# Autodesk Inventor assembly: ASY GBK предварительная торцевая
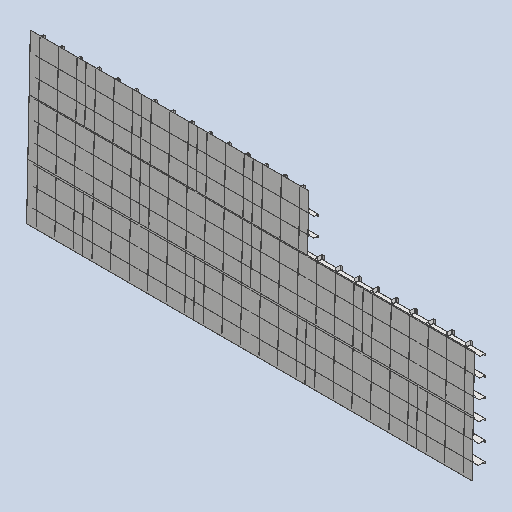
[picture p0: Inventor's stored thumbnail of the model, 512x512]
Saved by Autodesk Inventor 2026.2 (Build 302298000, 298)
## iProperties
Created: 2026-05-20
Part Number: ASY GBK предварительная торцевая
Document SubType Name: Assembly
Designer: admin
Mass: 2.96106e+06 g
Surface Area: 1.91261e+06 cm^2
Volume: 377205 cm^3
Density: 7.85 g/cm^3
Author: admin
## Documents named in this file (6)
- C:\Users\admin\Documents\Inventor\GBK-Gubkinskiy\ASY GBK предварительная торцевая.iam
- C:\Users\admin\Documents\Inventor\GBK-Gubkinskiy\ASY GBK 1110 long wall shield 1.iam
- C:\Users\admin\Documents\Inventor\GBK-Gubkinskiy\ASY GBK 1120 long wall shield 2.iam
- C:\Users\admin\Documents\Inventor\GBK-Gubkinskiy\ASY GBK 1210 long wall shield 3.iam
- C:\Users\admin\Documents\Inventor\GBK-Gubkinskiy\ASY GBK 1310 long wall shield 4.iam
- C:\Users\admin\Documents\Inventor\GBK-Gubkinskiy\08 ASY GBK wall shield 1.3.8.iam
## Components (14 placed, 5 different names)
1. ASY GBK 1110 long wall shield 1:1 [sub-assembly]
2. 02 ASY GBK wall shield 1.1.2:1 [sub-assembly]
3. 04 ASY GBK wall shield 1.2.4:1 [sub-assembly]
4. 07 ASY GBK wall shield 1.3.1:1 [sub-assembly]
5. 08 ASY GBK wall shield 1.3.8:1 [sub-assembly]
6. 08 ASY GBK wall shield 1.3.8:2 [sub-assembly]
7. 08 ASY GBK wall shield 1.3.8:3 [sub-assembly]
8. 04 ASY GBK wall shield 1.2.4:2 [sub-assembly]
9. 04 ASY GBK wall shield 1.2.4:3 [sub-assembly]
10. 04 ASY GBK wall shield 1.2.4:4 [sub-assembly]
11. 02 ASY GBK wall shield 1.1.2:2 [sub-assembly]
12. 02 ASY GBK wall shield 1.1.2:3 [sub-assembly]
13. 07 ASY GBK wall shield 1.3.1:2 [sub-assembly]
14. ASY GBK 1110 long wall shield 1:2 [sub-assembly]
## Relationships (13: WeldJoint 13)
- [WeldJoint] (1 mm): ASY GBK 1110 long wall shield 1:1 ↔ 02 ASY GBK wall shield 1.1.2:1
- [WeldJoint]: ASY GBK 1110 long wall shield 1:1 ↔ 04 ASY GBK wall shield 1.2.4:1
- [WeldJoint]: 04 ASY GBK wall shield 1.2.4:1 ↔ 07 ASY GBK wall shield 1.3.1:1
- [WeldJoint] (1 mm): 07 ASY GBK wall shield 1.3.1:1 ↔ 08 ASY GBK wall shield 1.3.8:1
- [WeldJoint] (1 mm): 08 ASY GBK wall shield 1.3.8:1 ↔ 08 ASY GBK wall shield 1.3.8:2
- [WeldJoint] (1 mm): 08 ASY GBK wall shield 1.3.8:2 ↔ 08 ASY GBK wall shield 1.3.8:3
- [WeldJoint] (1 mm): 04 ASY GBK wall shield 1.2.4:1 ↔ 04 ASY GBK wall shield 1.2.4:2
- [WeldJoint] (1 mm): 04 ASY GBK wall shield 1.2.4:2 ↔ 04 ASY GBK wall shield 1.2.4:3
- [WeldJoint] (1 mm): 04 ASY GBK wall shield 1.2.4:3 ↔ 04 ASY GBK wall shield 1.2.4:4
- [WeldJoint] (1 mm): 02 ASY GBK wall shield 1.1.2:1 ↔ 02 ASY GBK wall shield 1.1.2:2
- [WeldJoint] (1 mm): 02 ASY GBK wall shield 1.1.2:2 ↔ 02 ASY GBK wall shield 1.1.2:3
- [WeldJoint] (1 mm): 08 ASY GBK wall shield 1.3.8:3 ↔ 07 ASY GBK wall shield 1.3.1:2
- [WeldJoint] (1 mm): 02 ASY GBK wall shield 1.1.2:3 ↔ ASY GBK 1110 long wall shield 1:2
## Named parameters: d141_Зазор_по_горизонту = 1 mm, d142_d99 = 0 mm, d152_d98 = 0 mm
